# Autodesk Inventor assembly: GearBox_ProperConstraints
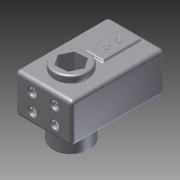
[picture p0: Inventor's stored thumbnail of the model, 180x180]
Saved by Autodesk Inventor 2012 (Build 160160000, 160)
## iProperties
Created: 2011-10-22
Part Number: GearBox_ProperConstraints
Document SubType Name: Assembly
Designer: KuttaA
Mass: 25.554 g
Surface Area: 211.568 cm^2
Volume: 25.554 cm^3
Density: 1 g/cm^3
Author: KuttaA
## Documents named in this file (7)
- C:\Users\Drew\Dropbox\Hexapod Research\Leg Design\Other Parts\Intermediary Gear Box\GearBox_ProperConstraints.iam
- C:\Users\Drew\Dropbox\Hexapod Research\Leg Design\Other Parts\Intermediary Gear Box\GearboxWallOutput.ipt
- C:\Users\Drew\Dropbox\Hexapod Research\Leg Design\Other Parts\Intermediary Gear Box\DerivedPartsFromAssemblies\LargeGearInput.ipt
- C:\Users\Drew\Dropbox\Hexapod Research\Leg Design\Other Parts\Intermediary Gear Box\DerivedPartsFromAssemblies\TransferGear.ipt
- C:\Users\Drew\Dropbox\Hexapod Research\Leg Design\Other Parts\Intermediary Gear Box\DerivedPartsFromAssemblies\SmallGearOutput.ipt
- C:\Users\Drew\Dropbox\Hexapod Research\Leg Design\Other Parts\Intermediary Gear Box\DerivedPartsFromAssemblies\GearboxTopAndAxle.ipt
- C:\Users\Drew\Dropbox\Hexapod Research\Leg Design\Other Parts\Intermediary Gear Box\GearBoxPin.ipt
## Components (9 placed, 6 different names)
1. GearboxWallOutput:1 — Mate:1, Mate:11, Mate:20, Mate:22, Mate:25, Mate:26, Mate:27, Mate:28, Mate:29, Mate:30, Flush:1, Flush:2, Flush:3, Flush:4, Mate:31, Mate:32
2. LargeGearInput:1 — Mate:11, Rotation:1, Mate:28
3. SmallGearOutput:1 — Mate:20, Mate:22, Rotation:2
4. TransferGear:1 — Rotation:1, Rotation:2, Mate:23, Mate:24
5. GearboxTopAndAxle:1 — Mate:23, Mate:24, Mate:25, Mate:26, Mate:27
6. GearBoxPin:1 — Flush:4, Mate:31
7. GearBoxPin:2 — Flush:3, Mate:32
8. GearBoxPin:3 — Mate:29, Flush:2
9. GearBoxPin:4 — Mate:30, Flush:1
## Relationships (20: Mate 14, Flush 4, RelateRotation 2)
- Mate:1: GearboxWallOutput:1
- Mate:11: GearboxWallOutput:1 ↔ LargeGearInput:1
- Mate:20: GearboxWallOutput:1 ↔ SmallGearOutput:1
- Mate:22 (0.3 mm): GearboxWallOutput:1 ↔ SmallGearOutput:1
- Rotation:1 [RelateRotation] (0.7692 ul): LargeGearInput:1 ↔ TransferGear:1
- Rotation:2 [RelateRotation] (1.3 ul): SmallGearOutput:1 ↔ TransferGear:1
- Mate:23: TransferGear:1 ↔ GearboxTopAndAxle:1
- Mate:24 (0.3 mm): TransferGear:1 ↔ GearboxTopAndAxle:1
- Mate:25 (0.3 mm): GearboxWallOutput:1 ↔ GearboxTopAndAxle:1
- Mate:26 (0.1 mm): GearboxWallOutput:1 ↔ GearboxTopAndAxle:1
- Mate:27: GearboxWallOutput:1 ↔ GearboxTopAndAxle:1
- Mate:28 (0.3 mm): GearboxWallOutput:1 ↔ LargeGearInput:1
- Mate:29: GearboxWallOutput:1 ↔ GearBoxPin:3
- Mate:30: GearboxWallOutput:1 ↔ GearBoxPin:4
- Flush:1: GearboxWallOutput:1 ↔ GearBoxPin:4
- Flush:2: GearboxWallOutput:1 ↔ GearBoxPin:3
- Flush:3: GearboxWallOutput:1 ↔ GearBoxPin:2
- Flush:4: GearboxWallOutput:1 ↔ GearBoxPin:1
- Mate:31: GearboxWallOutput:1 ↔ GearBoxPin:1
- Mate:32: GearboxWallOutput:1 ↔ GearBoxPin:2
